# Autodesk Inventor assembly: BBP
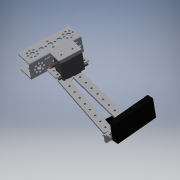
[picture p0: Inventor's stored thumbnail of the model, 180x180]
Saved by Autodesk Inventor 2016 (Build 200138000, 138)
## iProperties
Created: 2016-09-30
Part Number: BBP
Document SubType Name: Assembly
Designer: Delta
Author: Delta
## Documents named in this file (11)
- C:\Robotics\CAD\2016-17_CAD\BBP - Current.iam
- C:\Robotics\CAD\COTSParts\Tetrix\Tetrix channel 160mm.ipt
- C:\Robotics\CAD\COTSParts\Tetrix\Tetrix bracket - single servo.ipt
- C:\Robotics\CAD\COTSParts\Actobotics\585 parts\585382.ipt
- C:\Robotics\CAD\COTSParts\Tetrix\Tetrix servo 180.ipt
- C:\Robotics\CAD\2015-16_CAD\Part5.ipt
- C:\Robotics\CAD\2015-16_CAD\Part6.ipt
- C:\Robotics\CAD\2015-16_CAD\Tetrix angle 144mm_3in.ipt
- C:\Robotics\CAD\COTSParts\ModernRobotics\45-2006_ODS.ipt
- C:\Robotics\CAD\COTSParts\Tetrix\Tetrix flat bar 7 in.ipt
- C:\Robotics\CAD\COTSParts\Tetrix\Tetrix flat bar 5.75.ipt
## Components (11 placed, 10 different names)
1. Tetrix channel 160mm:2 — Insert:16, Insert:20
2. Tetrix bracket - single servo:1 — Mate:1, Flush:1, Flush:2, Insert:16
3. Tetrix servo 180:1 — Mate:1, Flush:1, Flush:2, Insert:21
4. 585382:5 — Insert:18, Mate:5, Flush:11, Flush:12, Mate:6
5. Part5:1 — Insert:19, Insert:20
6. Part6:1 — Mate:2, Flush:6, Flush:13
7. Tetrix angle 144mm_3in:1 — Flush:7, Flush:8, Mate:3, Flush:9, Flush:10, Flush:11, Flush:12, Mate:6
8. Tetrix angle 144mm_3in:2 — Mate:2, Flush:6, Flush:7, Flush:8, Mate:3, Flush:9, Flush:10, Flush:13
9. 45-2006_ODS:1 — Insert:22
10. Tetrix flat bar 7 in:1 — Insert:18, Insert:19, Insert:22
11. Tetrix flat bar 5.75:1 — Insert:21, Mate:5
## Relationships (21: Flush 10, Insert 6, Mate 5)
- Mate:1 (5.3594 mm): Tetrix bracket - single servo:1 ↔ Tetrix servo 180:1
- Flush:1: Tetrix bracket - single servo:1 ↔ Tetrix servo 180:1
- Flush:2: Tetrix bracket - single servo:1 ↔ Tetrix servo 180:1
- Mate:2: Part6:1 ↔ Tetrix angle 144mm_3in:2
- Flush:6: Part6:1 ↔ Tetrix angle 144mm_3in:2
- Flush:7: Tetrix angle 144mm_3in:1 ↔ Tetrix angle 144mm_3in:2
- Flush:8: Tetrix angle 144mm_3in:1 ↔ Tetrix angle 144mm_3in:2
- Mate:3: Tetrix angle 144mm_3in:1 ↔ Tetrix angle 144mm_3in:2
- Insert:16: Tetrix channel 160mm:2 ↔ Tetrix bracket - single servo:1
- Flush:9 (4.3434 mm): Tetrix angle 144mm_3in:1 ↔ Tetrix angle 144mm_3in:2
- Insert:18: 585382:5 ↔ Tetrix flat bar 7 in:1
- Insert:19: Part5:1 ↔ Tetrix flat bar 7 in:1
- Insert:20: Tetrix channel 160mm:2 ↔ Part5:1
- Insert:21: Tetrix servo 180:1 ↔ Tetrix flat bar 5.75:1
- Mate:5: 585382:5 ↔ Tetrix flat bar 5.75:1
- Flush:10: Tetrix angle 144mm_3in:1 ↔ Tetrix angle 144mm_3in:2
- Flush:11: 585382:5 ↔ Tetrix angle 144mm_3in:1
- Flush:12: 585382:5 ↔ Tetrix angle 144mm_3in:1
- Mate:6: 585382:5 ↔ Tetrix angle 144mm_3in:1
- Insert:22: 45-2006_ODS:1 ↔ Tetrix flat bar 7 in:1
- Flush:13: Part6:1 ↔ Tetrix angle 144mm_3in:2
